# Autodesk Inventor assembly: mg996r_right_rot_foot_servo
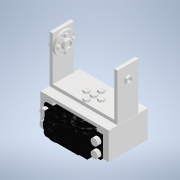
[picture p0: Inventor's stored thumbnail of the model, 180x180]
Saved by Autodesk Inventor 2021.4 (Build 254397000, 397)
## iProperties
Created: 2022-07-25
Part Number: mg996r_right_rot_foot_servo
Document SubType Name: Assembly
Designer: isamu
Author: isamu
## Documents named in this file (4)
- D:\personal_projects\robot\inventor\2021_matlab_compat _v2\motor_with_frames\mg996r_right_rot_foot_servo.iam
- D:\personal_projects\robot\inventor\2021_matlab_compat _v2\motor_with_frames\mg996r_top.iam
- D:\personal_projects\robot\inventor\2021_matlab_compat _v2\servo_rot_frame\mg996r_rot_frame.iam
- D:\personal_projects\robot\exports\screws\m3 nuts.ipt
## Components (7 placed, 3 different names)
1. mg996r_top:1 [sub-assembly] — Mate:1, Mate:2, Mate:3
2. mg996r_rot_frame:1 [sub-assembly] — Mate:1, Mate:2, Mate:3, Insert:1, Insert:2, Insert:3, Insert:4, Insert:5
3. m3 nuts:1 — Insert:4
4. m3 nuts:2 — Insert:2
5. m3 nuts:3 — Insert:1
6. m3 nuts:4 — Insert:3
7. m3 nuts:5 — Insert:5
## Relationships (8: Insert 5, Mate 3)
- Mate:1: mg996r_top:1 ↔ mg996r_rot_frame:1
- Mate:2: mg996r_top:1 ↔ mg996r_rot_frame:1
- Mate:3: mg996r_top:1 ↔ mg996r_rot_frame:1
- Insert:1: mg996r_rot_frame:1 ↔ m3 nuts:3
- Insert:2: mg996r_rot_frame:1 ↔ m3 nuts:2
- Insert:3: mg996r_rot_frame:1 ↔ m3 nuts:4
- Insert:4: mg996r_rot_frame:1 ↔ m3 nuts:1
- Insert:5: mg996r_rot_frame:1 ↔ m3 nuts:5
